# Autodesk Inventor assembly: BuchsenLeiste16
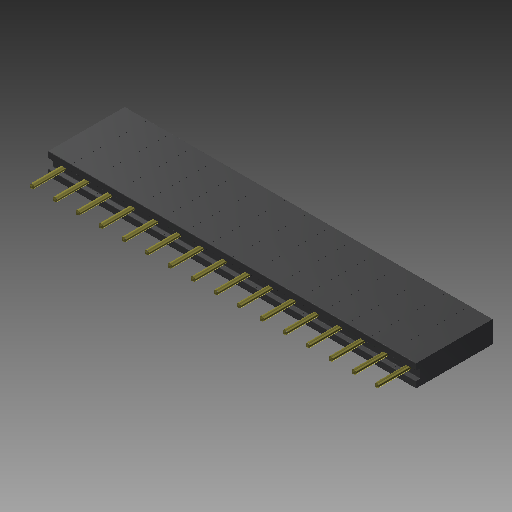
[picture p0: Inventor's stored thumbnail of the model, 512x512]
Saved by Autodesk Inventor 2017.3 (Build 213257000, 257)
## iProperties
Part Number: BuchsenLeiste16
Material: Generisch
Document SubType Name: Assembly
Designer: Enno
Author: Enno
## Documents named in this file (2)
- C:\Users\Enno-LT\Desktop\IMU_Motion_Classification\Casing\Stiftleiste\Weib\Gerade\BuchsenLeiste16.iam
- C:\Users\Enno-LT\Desktop\IMU_Motion_Classification\Casing\Stiftleiste\Weib\Gerade\Buchsenleiste_female.ipt
## Components (16 placed, 1 different names)
1. Buchsenleiste_female:17
2. Buchsenleiste_female:18
3. Buchsenleiste_female:19
4. Buchsenleiste_female:20
5. Buchsenleiste_female:21
6. Buchsenleiste_female:22
7. Buchsenleiste_female:23
8. Buchsenleiste_female:24
9. Buchsenleiste_female:25
10. Buchsenleiste_female:26
11. Buchsenleiste_female:27
12. Buchsenleiste_female:28 — Passend:75, Passend:76, Passend:77
13. Buchsenleiste_female:29 — Passend:75, Passend:76, Passend:77, Passend:78, Passend:79, Passend:80
14. Buchsenleiste_female:30 — Passend:78, Passend:79, Passend:80, Passend:81, Passend:82, Passend:83
15. Buchsenleiste_female:31 — Passend:81, Passend:82, Passend:83, Passend:84, Passend:85, Passend:86
16. Buchsenleiste_female:32 — Passend:84, Passend:85, Passend:86
## Relationships (45: Mate 45)
- [Mate]: Buchsenleiste_female:17 ↔ Buchsenleiste_female:18
- [Mate]: Buchsenleiste_female:17 ↔ Buchsenleiste_female:18
- [Mate]: Buchsenleiste_female:17 ↔ Buchsenleiste_female:18
- [Mate]: Buchsenleiste_female:18 ↔ Buchsenleiste_female:19
- [Mate]: Buchsenleiste_female:18 ↔ Buchsenleiste_female:19
- [Mate]: Buchsenleiste_female:18 ↔ Buchsenleiste_female:19
- [Mate]: Buchsenleiste_female:19 ↔ Buchsenleiste_female:20
- [Mate]: Buchsenleiste_female:19 ↔ Buchsenleiste_female:20
- [Mate]: Buchsenleiste_female:19 ↔ Buchsenleiste_female:20
- [Mate]: Buchsenleiste_female:20 ↔ Buchsenleiste_female:21
- [Mate]: Buchsenleiste_female:20 ↔ Buchsenleiste_female:21
- [Mate]: Buchsenleiste_female:20 ↔ Buchsenleiste_female:21
- [Mate]: Buchsenleiste_female:21 ↔ Buchsenleiste_female:22
- [Mate]: Buchsenleiste_female:21 ↔ Buchsenleiste_female:22
- [Mate]: Buchsenleiste_female:21 ↔ Buchsenleiste_female:22
- [Mate]: Buchsenleiste_female:22 ↔ Buchsenleiste_female:23
- [Mate]: Buchsenleiste_female:22 ↔ Buchsenleiste_female:23
- [Mate]: Buchsenleiste_female:22 ↔ Buchsenleiste_female:23
- [Mate]: Buchsenleiste_female:23 ↔ Buchsenleiste_female:24
- [Mate]: Buchsenleiste_female:23 ↔ Buchsenleiste_female:24
- [Mate]: Buchsenleiste_female:23 ↔ Buchsenleiste_female:24
- [Mate]: Buchsenleiste_female:24 ↔ Buchsenleiste_female:25
- [Mate]: Buchsenleiste_female:24 ↔ Buchsenleiste_female:25
- [Mate]: Buchsenleiste_female:24 ↔ Buchsenleiste_female:25
- [Mate]: Buchsenleiste_female:25 ↔ Buchsenleiste_female:26
- [Mate]: Buchsenleiste_female:25 ↔ Buchsenleiste_female:26
- [Mate]: Buchsenleiste_female:25 ↔ Buchsenleiste_female:26
- [Mate]: Buchsenleiste_female:26 ↔ Buchsenleiste_female:27
- [Mate]: Buchsenleiste_female:26 ↔ Buchsenleiste_female:27
- [Mate]: Buchsenleiste_female:26 ↔ Buchsenleiste_female:27
- [Mate]: Buchsenleiste_female:27 ↔ Buchsenleiste_female:28
- [Mate]: Buchsenleiste_female:27 ↔ Buchsenleiste_female:28
- [Mate]: Buchsenleiste_female:27 ↔ Buchsenleiste_female:28
- Passend:75 [Mate]: Buchsenleiste_female:28 ↔ Buchsenleiste_female:29
- Passend:76 [Mate]: Buchsenleiste_female:28 ↔ Buchsenleiste_female:29
- Passend:77 [Mate]: Buchsenleiste_female:28 ↔ Buchsenleiste_female:29
- Passend:78 [Mate]: Buchsenleiste_female:29 ↔ Buchsenleiste_female:30
- Passend:79 [Mate]: Buchsenleiste_female:29 ↔ Buchsenleiste_female:30
- Passend:80 [Mate]: Buchsenleiste_female:29 ↔ Buchsenleiste_female:30
- Passend:81 [Mate]: Buchsenleiste_female:30 ↔ Buchsenleiste_female:31
- Passend:82 [Mate]: Buchsenleiste_female:30 ↔ Buchsenleiste_female:31
- Passend:83 [Mate]: Buchsenleiste_female:30 ↔ Buchsenleiste_female:31
- Passend:84 [Mate]: Buchsenleiste_female:31 ↔ Buchsenleiste_female:32
- Passend:85 [Mate]: Buchsenleiste_female:31 ↔ Buchsenleiste_female:32
- Passend:86 [Mate]: Buchsenleiste_female:31 ↔ Buchsenleiste_female:32
## Named parameters: d45_d68 = 0 mm, d46_d69 = 0 mm, d47_d70 = 0 mm, d48_d71 = 0 mm, d49_d72 = 0 mm, d50_d73 = 0 mm, d51_d74 = 0 mm, d52_d75 = 0 mm, d53_d76 = 0 mm, d54_d77 = 0 mm, d55_d56 = 0 mm, d56_d57 = 0 mm, d57_d58 = 0 mm, d58_d59 = 0 mm, d59_d60 = 0 mm, d60_d61 = 0 mm, d61_d62 = 0 mm, d62_d63 = 0 mm, d63_d64 = 0 mm, d64_d65 = 0 mm, d65_d66 = 0 mm, d66_d67 = 0 mm
